# Autodesk Inventor assembly: Hori - Basic V0
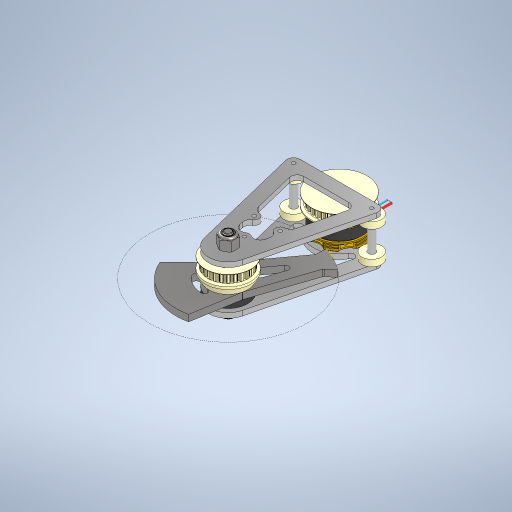
[picture p0: Inventor's stored thumbnail of the model, 512x512]
Saved by Autodesk Inventor 2023.4 (Build 274418000, 418)
## iProperties
Created: 2024-09-13
Part Number: Hori - Basic V0
Document SubType Name: Assembly
Designer: Nathan Cai
Mass: 559.5 g
Surface Area: 836.783 cm^2
Volume: 136.036 cm^3
Density: 4.11289 g/cm^3
Author: Nathan Cai
## Documents named in this file (14)
- E:\Documents\Inventor\Law - V2.1\Hori - Basic V0\Hori - Basic V0.iam
- E:\Documents\Inventor\Law - V2.1\Hori - Basic V0\Standoff 1.5in.ipt
- E:\Documents\Inventor\Law - V2.1\Hori - Basic V0\Upright - Motor.ipt
- E:\Documents\Inventor\Law - V2.1\Hori - Basic V0\Upright - Blank.ipt
- E:\Documents\Inventor\Law - V2.1\Hori - Basic V0\FEICHAO BE4108 380KV\FEICHAO BE4108 380KV.iam
- E:\Documents\Inventor\Law - V2.1\Hori - Basic V0\91259A632_Alloy Steel Shoulder Screw.ipt
- E:\Documents\Inventor\Law - V2.1\Hori - Basic V0\XL Pulley Base.ipt
- E:\Documents\Inventor\Law - V2.1\Hori - Basic V0\90630A121_High-Strength Steel Nylon-Insert Locknut.ipt
- E:\Documents\Inventor\Law - V2.1\Hori - Basic V0\Blade (Bar 3).ipt
- E:\Documents\Inventor\Law - V2.1\Hori - Basic V0\Needle Bearings.ipt
- E:\Documents\Inventor\Law - V2.1\Hori - Basic V0\5905K497_Needle-Roller Bearing (1).ipt
- E:\Documents\Inventor\Law - V2.1\Hori - Basic V0\Spacer 3-8x .125.ipt
- E:\Documents\Inventor\Law - V2.1\Hori - Basic V0\XL Pulley - Weapon.ipt
- E:\Documents\Inventor\Law - V2.1\Vert - Basic\STLs\Spacer.ipt
## Components (19 placed, 13 different names)
1. Upright - Motor:1 — Mate:1, Mate:2, Mate:3, Mate:4, Mate:5, Mate:6, Mate:7, Mate:8, Mate:9, Mate:10, Mate:11, Mate:12, Mate:24, Mate:37, Mate:41, Mate:42
2. Upright - Blank:1 — Mate:1, Mate:2, Mate:3, Mate:25, Mate:35, Mate:40
3. Standoff 1.5in:1 — Mate:5, Mate:7, Mate:34, Mate:36
4. Standoff 1.5in:2 — Mate:4, Mate:6, Mate:38, Mate:39
5. FEICHAO BE4108 380KV:1 [sub-assembly] — Mate:8, Mate:9, Mate:10, Mate:14, Mate:33
6. 91259A632_Alloy Steel Shoulder Screw:1 — Mate:11, Mate:12, Mate:15, Mate:16, Mate:17
7. XL Pulley Base:1 — Mate:14, Mate:29, Mate:33
8. 90630A121_High-Strength Steel Nylon-Insert Locknut:1 — Mate:15, Mate:16
9. Blade (Bar 3):1 — Mate:17, Mate:19, Mate:20, Mate:30, Mate:31, Mate:32
10. Needle Bearings:1 — Mate:22, Mate:23, Mate:24
11. Needle Bearings:2 — Mate:25, Mate:26, Mate:27
12. 5905K497_Needle-Roller Bearing (1):1 — Mate:18, Mate:27, Mate:28
13. 5905K497_Needle-Roller Bearing (1):2 — Mate:18, Mate:21, Flush:1, Mate:23
14. Spacer 3-8x .125:1 — Mate:19, Mate:20, Mate:21, Flush:1, Mate:22, Mate:26, Mate:31
15. XL Pulley - Weapon:1 — Mate:28, Mate:29, Mate:30, Mate:32
16. Spacer:1 — Mate:34, Mate:35
17. Spacer:2 — Mate:36, Mate:42
18. Spacer:3 — Mate:37, Mate:39, Mate:41
19. Spacer:4 — Mate:38, Mate:40
## Relationships (42: Mate 41, Flush 1)
- Mate:1 (38.1 mm): Upright - Motor:1 ↔ Upright - Blank:1
- Mate:2: Upright - Motor:1 ↔ Upright - Blank:1
- Mate:3: Upright - Motor:1 ↔ Upright - Blank:1
- Mate:4: Upright - Motor:1 ↔ Standoff 1.5in:2
- Mate:5: Upright - Motor:1 ↔ Standoff 1.5in:1
- Mate:6: Upright - Motor:1 ↔ Standoff 1.5in:2
- Mate:7: Upright - Motor:1 ↔ Standoff 1.5in:1
- Mate:8: Upright - Motor:1 ↔ FEICHAO BE4108 380KV:1
- Mate:9: Upright - Motor:1 ↔ FEICHAO BE4108 380KV:1
- Mate:10: Upright - Motor:1 ↔ FEICHAO BE4108 380KV:1
- Mate:11: Upright - Motor:1 ↔ 91259A632_Alloy Steel Shoulder Screw:1
- Mate:12 (3.175 mm): Upright - Motor:1 ↔ 91259A632_Alloy Steel Shoulder Screw:1
- Mate:14: FEICHAO BE4108 380KV:1 ↔ XL Pulley Base:1
- Mate:15: 91259A632_Alloy Steel Shoulder Screw:1 ↔ 90630A121_High-Strength Steel Nylon-Insert Locknut:1
- Mate:16: 91259A632_Alloy Steel Shoulder Screw:1 ↔ 90630A121_High-Strength Steel Nylon-Insert Locknut:1
- Mate:17: 91259A632_Alloy Steel Shoulder Screw:1 ↔ Blade (Bar 3):1
- Mate:18: 5905K497_Needle-Roller Bearing (1):1 ↔ 5905K497_Needle-Roller Bearing (1):2
- Mate:19: Blade (Bar 3):1 ↔ Spacer 3-8x .125:1
- Mate:20: Blade (Bar 3):1 ↔ Spacer 3-8x .125:1
- Mate:21: 5905K497_Needle-Roller Bearing (1):2 ↔ Spacer 3-8x .125:1
- Flush:1: 5905K497_Needle-Roller Bearing (1):2 ↔ Spacer 3-8x .125:1
- Mate:22: Needle Bearings:1 ↔ Spacer 3-8x .125:1
- Mate:23: Needle Bearings:1 ↔ 5905K497_Needle-Roller Bearing (1):2
- Mate:24: Upright - Motor:1 ↔ Needle Bearings:1
- Mate:25: Upright - Blank:1 ↔ Needle Bearings:2
- Mate:26: Needle Bearings:2 ↔ Spacer 3-8x .125:1
- Mate:27: Needle Bearings:2 ↔ 5905K497_Needle-Roller Bearing (1):1
- Mate:28: 5905K497_Needle-Roller Bearing (1):1 ↔ XL Pulley - Weapon:1
- Mate:29: XL Pulley Base:1 ↔ XL Pulley - Weapon:1
- Mate:30: Blade (Bar 3):1 ↔ XL Pulley - Weapon:1
- Mate:31: Blade (Bar 3):1 ↔ Spacer 3-8x .125:1
- Mate:32: Blade (Bar 3):1 ↔ XL Pulley - Weapon:1
- Mate:33: FEICHAO BE4108 380KV:1 ↔ XL Pulley Base:1
- Mate:34: Standoff 1.5in:1 ↔ Spacer:1
- Mate:35: Upright - Blank:1 ↔ Spacer:1
- Mate:36: Standoff 1.5in:1 ↔ Spacer:2
- Mate:37: Upright - Motor:1 ↔ Spacer:3
- Mate:38: Standoff 1.5in:2 ↔ Spacer:4
- Mate:39: Standoff 1.5in:2 ↔ Spacer:3
- Mate:40: Upright - Blank:1 ↔ Spacer:4
- Mate:41: Upright - Motor:1 ↔ Spacer:3
- Mate:42: Upright - Motor:1 ↔ Spacer:2
